# Autodesk Inventor assembly: ensembleFinal
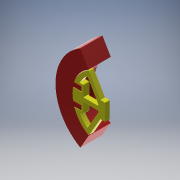
[picture p0: Inventor's stored thumbnail of the model, 180x180]
Saved by Autodesk Inventor 2019 (Build 230136000, 136)
## iProperties
Created: 2021-01-15
Part Number: ensembleFinal
Material: Générique
Document SubType Name: Assembly
Designer: tom.mousset
Author: tom.mousset
## Documents named in this file (3)
- F:\triSmarties\ensembleFinal.iam
- F:\triSmarties\pieceMere.ipt
- F:\triSmarties\bacRecupBonbon.ipt
## Components (2 placed, 2 different names)
1. pieceMere:1 — Placage:1, Affleurement:1, Affleurement:2
2. bacRecupBonbon:1 — Placage:1, Affleurement:1, Affleurement:2
## Relationships (3: Flush 2, Mate 1)
- Placage:1 [Mate]: pieceMere:1 ↔ bacRecupBonbon:1
- Affleurement:1 [Flush]: pieceMere:1 ↔ bacRecupBonbon:1
- Affleurement:2 [Flush]: pieceMere:1 ↔ bacRecupBonbon:1
